# Autodesk Inventor assembly: Right Rear Wheel with hub shaft and pulley
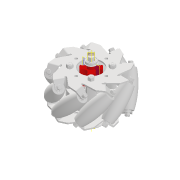
[picture p0: Inventor's stored thumbnail of the model, 180x180]
Saved by Autodesk Inventor 2020 (Build 240168000, 168)
## iProperties
Created: 2020-02-22
Part Number: Right Rear Wheel with hub shaft and pulley
Document SubType Name: Assembly
Designer: ball
Author: ball
## Documents named in this file (7)
- C:\FTC\FTC8863CAD\2019 Robot\Mecanum Drive Train Metal\Right Rear Wheel with hub shaft and pulley.iam
- C:\FTC\FTC8863CAD\2019 Robot\Mecanum Drive Train Metal\Right Rear Wheel with hub.iam
- C:\FTC\FTC8863CAD\GoBilda\2102 Parts\2102-0008-0090.ipt
- C:\FTC\FTC8863CAD\GoBilda\3414 Parts\3414-4008-0016 assembly.iam
- C:\FTC\FTC8863CAD\2019 Robot\Mecanum Drive Train Metal\wheel spacer for bearing.ipt
- C:\FTC\FTC8863CAD\GoBilda\1601 Parts\1601-0014-0008.ipt
- C:\FTC\FTC8863CAD\GoBilda\2807 Parts\2807-0811-0500.ipt
## Components (7 placed, 6 different names)
1. Right Rear Wheel with hub:1 [sub-assembly] — Flush:1, Mate:1, Mate:2, Mate:4, Mate:6
2. 2102-0008-0090:1 — Flush:1, Mate:1, Mate:2, Mate:3, Mate:5, Mate:7, Angle:1, Mate:8, Mate:11, Mate:13
3. 3414-4008-0016 assembly:1 [sub-assembly] — Mate:3, Mate:4, Mate:5, Mate:10
4. wheel spacer for bearing:1 — Mate:6, Mate:7, Angle:1, Mate:9
5. 1601-0014-0008:1 — Mate:8, Mate:9
6. 1601-0014-0008:2 — Mate:12, Mate:13
7. 2807-0811-0500:1 — Mate:10, Mate:11, Mate:12
## Relationships (15: Mate 13, Flush 1, Angle 1)
- Flush:1 (-17.1704 mm): Right Rear Wheel with hub:1 ↔ 2102-0008-0090:1
- Mate:1: Right Rear Wheel with hub:1 ↔ 2102-0008-0090:1
- Mate:2: Right Rear Wheel with hub:1 ↔ 2102-0008-0090:1
- Mate:3: 2102-0008-0090:1 ↔ 3414-4008-0016 assembly:1
- Mate:4: Right Rear Wheel with hub:1 ↔ 3414-4008-0016 assembly:1
- Mate:5: 2102-0008-0090:1 ↔ 3414-4008-0016 assembly:1
- Mate:6: Right Rear Wheel with hub:1 ↔ wheel spacer for bearing:1
- Mate:7: 2102-0008-0090:1 ↔ wheel spacer for bearing:1
- Angle:1 (45 deg): 2102-0008-0090:1 ↔ wheel spacer for bearing:1
- Mate:8: 2102-0008-0090:1 ↔ 1601-0014-0008:1
- Mate:9: wheel spacer for bearing:1 ↔ 1601-0014-0008:1
- Mate:10: 3414-4008-0016 assembly:1 ↔ 2807-0811-0500:1
- Mate:11: 2102-0008-0090:1 ↔ 2807-0811-0500:1
- Mate:12: 1601-0014-0008:2 ↔ 2807-0811-0500:1
- Mate:13: 2102-0008-0090:1 ↔ 1601-0014-0008:2
